# Autodesk Inventor assembly: 109
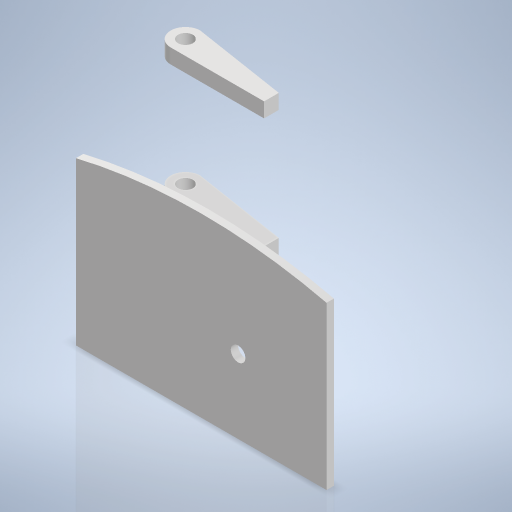
[picture p0: Inventor's stored thumbnail of the model, 512x512]
Saved by Autodesk Inventor 2024 (Build 280153000, 153)
## iProperties
Created: 2024-07-24
Part Number: 109
Document SubType Name: Assembly
Designer: ffogue
Author: ffogue
## Documents named in this file (3)
- C:\Users\ffogue\OneDrive - MuM - OM\Dokumente\Inventor\Freedom\109.iam
- C:\Users\ffogue\OneDrive - MuM - OM\Dokumente\Inventor\Freedom\MS.ipt
- C:\Users\ffogue\OneDrive - MuM - OM\Dokumente\Inventor\Freedom\109 part 2.ipt
## Components (3 placed, 2 different names)
1. MS:1
2. 109 part 2:1 — Passend:1
3. 109 part 2:2 — Passend:1
## Relationships (1: Mate 1)
- Passend:1 [Mate]: 109 part 2:1 ↔ 109 part 2:2
